# Autodesk Inventor assembly: Dexoay
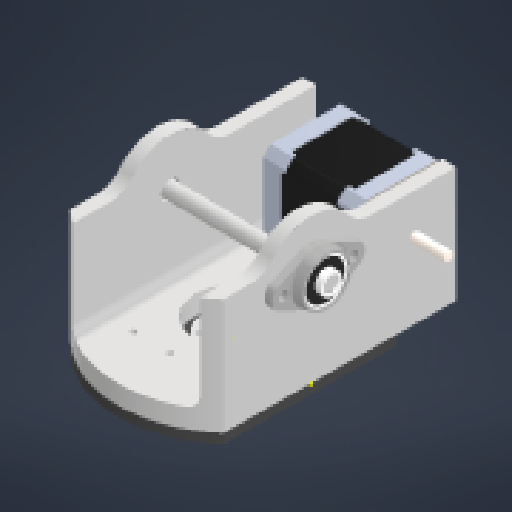
[picture p0: Inventor's stored thumbnail of the model, 512x512]
Saved by Autodesk Inventor 2023 (Build 270158000, 158)
## iProperties
Created: 2023-09-09
Part Number: Dexoay
Document SubType Name: Assembly
Designer: philo
Author: philo
## Documents named in this file (11)
- C:\Users\philo\OneDrive\Desktop\HK1-2024\TT ROBOT\02_3D_design_new\Dexoay.iam
- C:\Users\philo\OneDrive\Desktop\HK1-2024\TT ROBOT\02_3D_design_new\Diaquay.ipt
- C:\Users\philo\OneDrive\Desktop\HK1-2024\TT ROBOT\02_3D_design_new\goidoObi.ipt
- C:\Users\philo\OneDrive\Desktop\HK1-2024\TT ROBOT\02_3D_design_new\truc8mmew.ipt
- C:\Users\philo\OneDrive\Desktop\HK1-2024\TT ROBOT\02_3D_design_new\Part1.ipt
- C:\Users\philo\OneDrive\Desktop\HK1-2024\TT ROBOT\02_3D_design_new\codinhtruc.ipt
- C:\Users\philo\OneDrive\Desktop\HK1-2024\TT ROBOT\02_3D_design\STEP MOTOR NEMA 17.ipt
- C:\Users\philo\OneDrive\Desktop\HK1-2024\TT ROBOT\02_3D_design\GT2 Pulley 20 Tooth (ID6mm).ipt
- C:\Users\philo\OneDrive\Desktop\HK1-2024\TT ROBOT\02_3D_design_new\60pitch pulley GT2 6mm ASSEMBLY.iam
- C:\Users\philo\OneDrive\Desktop\HK1-2024\TT ROBOT\02_3D_design_new\limitswitch.ipt
- C:\Users\philo\OneDrive\Desktop\HK1-2024\TT ROBOT\02_3D_design_new\thanhdolimit.ipt
## Components (11 placed, 10 different names)
1. Diaquay:1 — Flush:1, Mate:3, Mate:4
2. goidoObi:1
3. goidoObi:2 — Mate:7, Mate:9
4. truc8mmew:1 — Flush:5, Mate:7, Mate:8, Flush:6, Mate:10
5. Part1:1 — Mate:1, Flush:1, Mate:2, Mate:3, Mate:4, Flush:2, Flush:3, Flush:5, Mate:9, Mate:10, Flush:7, Flush:8, Flush:9, Flush:10
6. codinhtruc:1 — Mate:2
7. STEP MOTOR NEMA 17:1 — Mate:1, Flush:2, Flush:3, Mate:5, Flush:4, Mate:11
8. GT2 Pulley 20 Tooth (ID6mm):1 — Mate:5, Flush:4
9. 60pitch pulley GT2 6mm ASSEMBLY:1 [sub-assembly] — Mate:8, Flush:6
10. limitswitch:1 — Flush:7, Mate:11, Mate:12, Mate:13, Mate:14
11. thanhdolimit:1 — Flush:8, Flush:9, Mate:12, Mate:13, Mate:14, Flush:10
## Relationships (23: Mate 13, Flush 10)
- Mate:1: Part1:1 ↔ STEP MOTOR NEMA 17:1
- Flush:1: Diaquay:1 ↔ Part1:1
- Mate:2: Part1:1 ↔ codinhtruc:1
- Mate:3: Diaquay:1 ↔ Part1:1
- Mate:4: Diaquay:1 ↔ Part1:1
- Flush:2: Part1:1 ↔ STEP MOTOR NEMA 17:1
- Flush:3: Part1:1 ↔ STEP MOTOR NEMA 17:1
- Mate:5: STEP MOTOR NEMA 17:1 ↔ GT2 Pulley 20 Tooth (ID6mm):1
- Flush:4 (-3 mm): STEP MOTOR NEMA 17:1 ↔ GT2 Pulley 20 Tooth (ID6mm):1
- Flush:5 (-30 mm): truc8mmew:1 ↔ Part1:1
- Mate:7: goidoObi:2 ↔ truc8mmew:1
- Mate:8: truc8mmew:1 ↔ 60pitch pulley GT2 6mm ASSEMBLY:1
- Flush:6: truc8mmew:1 ↔ 60pitch pulley GT2 6mm ASSEMBLY:1
- Mate:9: goidoObi:2 ↔ Part1:1
- Mate:10: truc8mmew:1 ↔ Part1:1
- Flush:7 (25 mm): Part1:1 ↔ limitswitch:1
- Mate:11 (5 mm): STEP MOTOR NEMA 17:1 ↔ limitswitch:1
- Flush:8: Part1:1 ↔ thanhdolimit:1
- Flush:9: Part1:1 ↔ thanhdolimit:1
- Mate:12: limitswitch:1 ↔ thanhdolimit:1
- Mate:13: limitswitch:1 ↔ thanhdolimit:1
- Mate:14: limitswitch:1 ↔ thanhdolimit:1
- Flush:10: Part1:1 ↔ thanhdolimit:1
